# Autodesk Inventor assembly: mount3
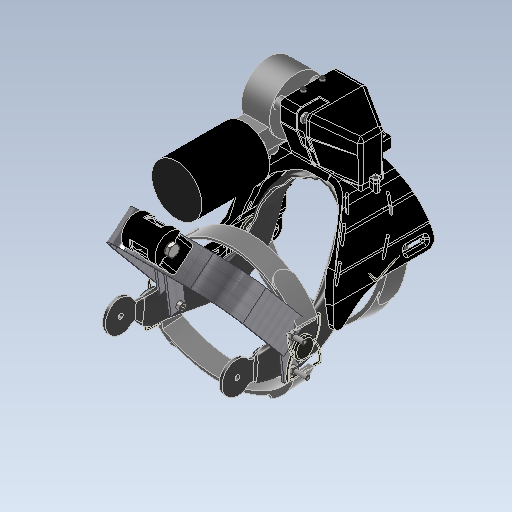
[picture p0: Inventor's stored thumbnail of the model, 512x512]
Saved by Autodesk Inventor 2025.2 (Build 292293000, 293)
## iProperties
Created: 2025-02-11
Part Number: mount3
Document SubType Name: Assembly
Designer: Alex
Author: Alex
## Documents named in this file (21)
- C:\Users\email\Desktop\Projects\Capstone\4TB6\CAD_Model\thigh_mount_2\thighmount_assembly_2.1.iam
- C:\Users\email\Desktop\Projects\Capstone\4TB6\CAD_Model\thigh_mount_2\thigh.ipt
- C:\Users\email\Desktop\Projects\Capstone\4TB6\CAD_Model\thigh_mount_2\thighmount2.1.ipt
- C:\Users\email\Desktop\Projects\Capstone\4TB6\CAD_Model\thigh_mount_2\motor.ipt
- C:\Users\email\Desktop\Projects\Capstone\4TB6\CAD_Model\thigh_mount_2\spool_temp.ipt
- C:\Users\email\Desktop\Projects\Capstone\4TB6\CAD_Model\thigh_mount_2\magnetholder.ipt
- C:\Users\email\Desktop\Projects\Capstone\4TB6\CAD_Model\thigh_mount_2\imu_house_assembly.iam
- C:\Users\email\Desktop\Projects\Capstone\4TB6\CAD_Model\thigh_mount_2\as5600mount_2.ipt
- C:\Users\email\Desktop\Projects\Capstone\4TB6\CAD_Model\thigh_mount_2\pulley_bracket_assem.iam
- C:\Users\email\Desktop\Projects\Capstone\4TB6\CAD_Model\thigh_mount_2\brace_tabs.ipt
- C:\Users\email\Desktop\Projects\Capstone\4TB6\CAD_Model\thigh_mount_2\brace_tabs_half.ipt
- C:\Users\email\Desktop\Projects\Capstone\4TB6\CAD_Model\thigh_mount_2\short_L_bracket.ipt
- C:\Users\email\Desktop\Projects\Capstone\4TB6\CAD_Model\thigh_mount_2\fasteners\AS 1420 - 1973 - M3 x 6.ipt
- C:\Users\email\Documents\Inventor\Content Center Files\R2025\en-US\AS 1420\AS 1420 - 1973 - M6 x 30.ipt
- C:\Users\email\Documents\Inventor\Content Center Files\R2025\en-US\AS 1420\AS 1420 - 1973 - M5 x 10.ipt
- C:\Users\email\Desktop\Projects\Capstone\4TB6\CAD_Model\thigh_mount_2\as5600.ipt
- C:\Users\email\Desktop\Projects\Capstone\4TB6\CAD_Model\thigh_mount_2\cover.ipt
- C:\Users\email\Desktop\Projects\Capstone\4TB6\CAD_Model\thigh_mount_2\spool_blocker.ipt
- C:\Users\email\Desktop\Projects\Capstone\4TB6\CAD_Model\thigh_mount_2\thigh_strap_01.ipt
- C:\Users\email\Desktop\Projects\Capstone\4TB6\CAD_Model\thigh_mount_2\thigh_strap_02.ipt
- C:\Users\email\Desktop\Projects\Capstone\4TB6\CAD_Model\thigh_mount_2\thigh_strap_03.ipt
## Components (36 placed, 20 different names)
1. thigh:1 — Mate:1, Mate:2, Flush:1, Mate:28, Mate:29, Mate:30, Mate:31, Mate:32, Mate:33
2. thighmount2.1:1 — Flush:4, Mate:5, Angle:7, Angle:2, Mate:21, Mate:22, Angle:8, Flush:5, Rigid:3, Rigid:4, Flush:7, Mate:38, Mate:39, Mate:40, Mate:41, Mate:49, Mate:50, Angle:9, Mate:51, Mate:52
3. motor:1 — Mate:5, Mate:7, Mate:23, Mate:48, Mate:53, Mate:54
4. spool_temp:1 — Mate:7, Mate:9, Mate:10, Mate:11, Mate:23, Mate:48
5. magnetholder:1 — Mate:9, Mate:10, Mate:11, Rotational:2, Rigid:5, Mate:47
6. imu_house_assembly:1 [sub-assembly] — Angle:8, Flush:5, Mate:51, Rigid:11
7. pulley_bracket_assem:1 [sub-assembly] — Angle:7, Angle:2, Mate:21, Mate:22
8. brace_tabs:1 — Mate:28, Mate:29
9. brace_tabs:2 — Mate:30, Mate:31
10. brace_tabs_half:1 — Mate:32
11. brace_tabs_half:2 — Mate:33
12. brace_tabs_half:3
13. short_L_bracket:1 — Rigid:10
14. AS 1420 - Metric M5 x 10:1 — Rigid:10
15. AS 1420 - Metric M6 x 30:1
16. AS 1420 - Metric M3 x 6:1 — Insert:7
17. AS 1420 - Metric M3 x 6:2 — Insert:6
18. AS 1420 - Metric M3 x 6:3 — Rigid:11
19. AS 1420 - Metric M6 x 30:2 — Rigid:4, Mate:54
20. AS 1420 - Metric M6 x 30:3 — Rigid:3, Mate:53
21. AS 1420 - Metric M3 x 6:4 — Rotational:2
22. AS 1420 - Metric M3 x 6:5 — Rigid:5
23. as5600:1 — Rotational:3, Rotational:4, Rotational:5, Rigid:6, Mate:46
24. AS 1420 - Metric M3 x 6:6 — Rotational:3
25. AS 1420 - Metric M3 x 6:7 — Rotational:4, Mate:44
26. AS 1420 - Metric M3 x 6:8 — Rotational:5, Mate:45
27. AS 1420 - Metric M3 x 6:9 — Rigid:6
28. cover:1 — Flush:7, Mate:38, Mate:39, Mate:40, Rigid:7, Rigid:8, Rigid:9
29. AS 1420 - Metric M3 x 6:10 — Rigid:7
30. AS 1420 - Metric M3 x 6:11 — Rigid:9
31. AS 1420 - Metric M3 x 6:12 — Rigid:8
32. as5600mount_2:1 — Mate:41, Mate:44, Mate:45, Mate:46, Mate:47, Insert:6, Insert:7
33. spool_blocker:1 — Mate:49, Mate:50, Angle:9
34. thigh_strap_01:1 — Flush:8
35. thigh_strap_02:1
36. thigh_strap_03:1 — Mate:52, Flush:8
## Relationships (56: Mate 31, WeldJoint 9, Flush 6, Angle 4, RevoluteJoint 4, Insert 2)
- Mate:1: thigh:1
- Mate:2: thigh:1
- Flush:1: thigh:1
- Flush:3 (-15 mm)
- Flush:4: thighmount2.1:1
- Mate:5: thighmount2.1:1 ↔ motor:1
- Mate:7: motor:1 ↔ spool_temp:1
- Mate:9: spool_temp:1 ↔ magnetholder:1
- Mate:10: spool_temp:1 ↔ magnetholder:1
- Mate:11: spool_temp:1 ↔ magnetholder:1
- Angle:7 (0 deg): thighmount2.1:1 ↔ pulley_bracket_assem:1
- Angle:2 (-40 deg): thighmount2.1:1 ↔ pulley_bracket_assem:1
- Mate:21 (-30 mm): thighmount2.1:1 ↔ pulley_bracket_assem:1
- Mate:22 (-40 mm): thighmount2.1:1 ↔ pulley_bracket_assem:1
- Mate:23: motor:1 ↔ spool_temp:1
- Mate:28: thigh:1 ↔ brace_tabs:1
- Mate:29: thigh:1 ↔ brace_tabs:1
- Mate:30: thigh:1 ↔ brace_tabs:2
- Mate:31: thigh:1 ↔ brace_tabs:2
- Mate:32: thigh:1 ↔ brace_tabs_half:1
- Mate:33 (2 mm): thigh:1 ↔ brace_tabs_half:2
- Angle:8 (90 deg): thighmount2.1:1 ↔ imu_house_assembly:1
- Flush:5: thighmount2.1:1 ↔ imu_house_assembly:1
- Rigid:3 [WeldJoint]: thighmount2.1:1 ↔ AS 1420 - Metric M6 x 30:3
- Rigid:4 [WeldJoint]: thighmount2.1:1 ↔ AS 1420 - Metric M6 x 30:2
- Rotational:2 [RevoluteJoint]: magnetholder:1 ↔ AS 1420 - Metric M3 x 6:4
- Rigid:5 [WeldJoint]: magnetholder:1 ↔ AS 1420 - Metric M3 x 6:5
- Rotational:3 [RevoluteJoint]: as5600:1 ↔ AS 1420 - Metric M3 x 6:6
- Rotational:4 [RevoluteJoint]: as5600:1 ↔ AS 1420 - Metric M3 x 6:7
- Rotational:5 [RevoluteJoint]: as5600:1 ↔ AS 1420 - Metric M3 x 6:8
- Rigid:6 [WeldJoint]: as5600:1 ↔ AS 1420 - Metric M3 x 6:9
- Flush:7: thighmount2.1:1 ↔ cover:1
- Mate:38: thighmount2.1:1 ↔ cover:1
- Mate:39: thighmount2.1:1 ↔ cover:1
- Mate:40: thighmount2.1:1 ↔ cover:1
- Rigid:7 [WeldJoint]: cover:1 ↔ AS 1420 - Metric M3 x 6:10
- Rigid:8 [WeldJoint]: cover:1 ↔ AS 1420 - Metric M3 x 6:12
- Rigid:9 [WeldJoint]: cover:1 ↔ AS 1420 - Metric M3 x 6:11
- Mate:41: thighmount2.1:1 ↔ as5600mount_2:1
- Mate:44: AS 1420 - Metric M3 x 6:7 ↔ as5600mount_2:1
- Mate:45: AS 1420 - Metric M3 x 6:8 ↔ as5600mount_2:1
- Mate:46: as5600:1 ↔ as5600mount_2:1
- Mate:47: magnetholder:1 ↔ as5600mount_2:1
- Mate:48: motor:1 ↔ spool_temp:1
- Insert:6: AS 1420 - Metric M3 x 6:2 ↔ as5600mount_2:1
- Insert:7: AS 1420 - Metric M3 x 6:1 ↔ as5600mount_2:1
- Rigid:10 [WeldJoint]: short_L_bracket:1 ↔ AS 1420 - Metric M5 x 10:1
- Mate:49: thighmount2.1:1 ↔ spool_blocker:1
- Mate:50: thighmount2.1:1 ↔ spool_blocker:1
- Angle:9 (90 deg): thighmount2.1:1 ↔ spool_blocker:1
- Mate:51: thighmount2.1:1 ↔ imu_house_assembly:1
- Rigid:11 [WeldJoint]: imu_house_assembly:1 ↔ AS 1420 - Metric M3 x 6:3
- Mate:52: thighmount2.1:1 ↔ thigh_strap_03:1
- Flush:8: thigh_strap_01:1 ↔ thigh_strap_03:1
- Mate:53: motor:1 ↔ AS 1420 - Metric M6 x 30:3
- Mate:54: motor:1 ↔ AS 1420 - Metric M6 x 30:2
